# Autodesk Inventor assembly: stojak
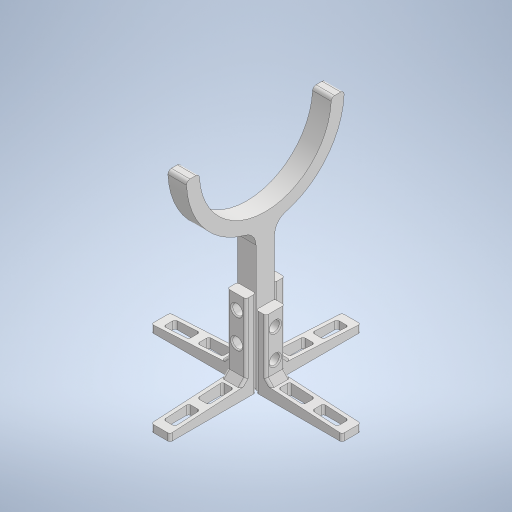
[picture p0: Inventor's stored thumbnail of the model, 512x512]
Saved by Autodesk Inventor 2024.2 (Build 282272000, 272)
## iProperties
Created: 2024-06-19
Part Number: stojak
Document SubType Name: Assembly
Designer: Konrad
Author: Konrad
## Documents named in this file (4)
- D:\Inventor\magisterka\akcesoria_czujnika\stojak.iam
- D:\Inventor\magisterka\akcesoria_czujnika\noga1.ipt
- D:\Inventor\magisterka\akcesoria_czujnika\noga2.ipt
- D:\Inventor\magisterka\akcesoria_czujnika\stojak.ipt
## Components (5 placed, 3 different names)
1. noga1:1 — Zestawiające:10, Zestawiające:11, Zestawiające:12
2. noga2:1 — Zestawiające:1, Zestawiające:2, Zestawiające:3, Zestawiające:4
3. stojak:1 — Zestawiające:2, Zestawiające:3, Zestawiające:4, Zestawiające:5, Zestawiające:6, Zestawiające:7, Zestawiające:8, Zestawiające:9, Zestawiające:10, Zestawiające:11, Zestawiające:12
4. noga2:2 — Zestawiające:5, Zestawiające:6
5. noga1:2 — Zestawiające:7, Zestawiające:8, Zestawiające:9
## Relationships (12: Mate 12)
- Zestawiające:1 [Mate]: noga2:1
- Zestawiające:2 [Mate]: noga2:1 ↔ stojak:1
- Zestawiające:3 [Mate]: noga2:1 ↔ stojak:1
- Zestawiające:4 [Mate]: noga2:1 ↔ stojak:1
- Zestawiające:5 [Mate]: stojak:1 ↔ noga2:2
- Zestawiające:6 [Mate]: stojak:1 ↔ noga2:2
- Zestawiające:7 [Mate]: stojak:1 ↔ noga1:2
- Zestawiające:8 [Mate]: stojak:1 ↔ noga1:2
- Zestawiające:9 [Mate]: stojak:1 ↔ noga1:2
- Zestawiające:10 [Mate]: noga1:1 ↔ stojak:1
- Zestawiające:11 [Mate]: noga1:1 ↔ stojak:1
- Zestawiające:12 [Mate]: noga1:1 ↔ stojak:1
